# Autodesk Inventor assembly: Zlozenie_na_igle_z_nakretka
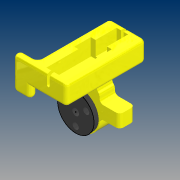
[picture p0: Inventor's stored thumbnail of the model, 180x180]
Saved by Autodesk Inventor 2021 (Build 250183000, 183)
## iProperties
Created: 2022-10-07
Part Number: Zlozenie_na_igle_z_nakretka
Document SubType Name: Assembly
Designer: agnpi
Author: agnpi
## Documents named in this file (3)
- E:\Users\agnpi\Desktop\lekcje\SEMESTR VII\Inventor inzynierka\Zlozenie_na_igle_z_nakretka.iam
- E:\Users\agnpi\Desktop\lekcje\SEMESTR VII\Inventor inzynierka\uchwyt_na_igle_.ipt
- E:\Users\agnpi\Desktop\lekcje\SEMESTR VII\Inventor inzynierka\Nakretka_na_igle_.ipt
## Components (2 placed, 2 different names)
1. uchwyt_na_igle_:1 — Mate:1, Mate:2, Mate:3, Mate:4, Mate:5
2. Nakretka_na_igle_:1 — Mate:1, Mate:2, Mate:3, Mate:4, Mate:5
## Relationships (5: Mate 5)
- Mate:1: uchwyt_na_igle_:1 ↔ Nakretka_na_igle_:1
- Mate:2: uchwyt_na_igle_:1 ↔ Nakretka_na_igle_:1
- Mate:3: uchwyt_na_igle_:1 ↔ Nakretka_na_igle_:1
- Mate:4: uchwyt_na_igle_:1 ↔ Nakretka_na_igle_:1
- Mate:5: uchwyt_na_igle_:1 ↔ Nakretka_na_igle_:1
